# Autodesk Inventor assembly: 組合檔
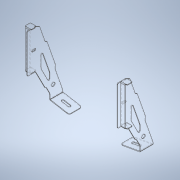
[picture p0: Inventor's stored thumbnail of the model, 180x180]
Saved by Autodesk Inventor 2020 (Build 240168000, 168)
## iProperties
Created: 2015-11-28
Part Number: 組合檔
Document SubType Name: Assembly
Designer: 設計製圖
Author: 設計製圖
## Documents named in this file (5)
- D:\資料庫\設計-3D Project\【May club 】\得利卡-車頂燈架\模型、圖面\短-車頂燈架-組合(#11.02)- 組合件1.iam
- D:\資料庫\設計-3D Project\【May club 】\得利卡-車頂燈架\模型、圖面\焊接組件-1(#11.02).ipt
- D:\資料庫\設計-3D Project\【May club 】\得利卡-車頂燈架\模型、圖面\吊架-短(R)(#11.02).ipt
- D:\資料庫\設計-3D Project\【May club 】\得利卡-車頂燈架\模型、圖面\吊架-短(L)(#11.02)_MIR.ipt
- D:\資料庫\設計-3D Project\【May club 】\得利卡-車頂燈架\模型、圖面\焊接組件-1(#11.02)_MIR.ipt
## Components (4 placed, 4 different names)
1. 吊架-短(R)(#11.02):1 — 貼合:23, 貼合:26, 齊平:18, 齊平:19
2. 焊接組件-1(#11.02):1 — 貼合:23, 貼合:26, 齊平:18
3. 吊架-短(L)(#11.02)_MIR:1 — 貼合:29
4. 焊接組件-1(#11.02)_MIR:1
## Relationships (5: Mate 3, Flush 2)
- 貼合:23 [Mate]: 吊架-短(R)(#11.02):1 ↔ 焊接組件-1(#11.02):1
- 貼合:26 [Mate]: 吊架-短(R)(#11.02):1 ↔ 焊接組件-1(#11.02):1
- 齊平:18 [Flush]: 吊架-短(R)(#11.02):1 ↔ 焊接組件-1(#11.02):1
- 齊平:19 [Flush] (150 mm): 吊架-短(R)(#11.02):1
- 貼合:29 [Mate] (150 mm): 吊架-短(L)(#11.02)_MIR:1
